# Autodesk Inventor assembly: Plastic Gear Test
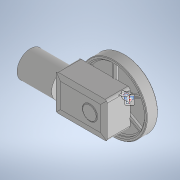
[picture p0: Inventor's stored thumbnail of the model, 180x180]
Saved by Autodesk Inventor 2020.2 (Build 242310000, 310)
## iProperties
Created: 2020-04-13
Part Number: Plastic Gear Test
Document SubType Name: Assembly
Designer: Josiah
Author: Josiah
## Documents named in this file (3)
- C:\Users\josia\OneDrive\Apps\0011_VentControlValve\Plastic Gear Test.iam
- C:\Users\josia\OneDrive\Apps\0011_VentControlValve\motor+Gearbox.ipt
- C:\Users\josia\OneDrive\Apps\0011_VentControlValve\Test Gear.ipt
## Components (2 placed, 2 different names)
1. motor+Gearbox:1 — Flush:1, Mate:1, Angle:1
2. Test Gear:1 — Flush:1, Mate:1, Angle:1
## Relationships (3: Flush 1, Mate 1, Angle 1)
- Flush:1: motor+Gearbox:1 ↔ Test Gear:1
- Mate:1: motor+Gearbox:1 ↔ Test Gear:1
- Angle:1 (180 deg): motor+Gearbox:1 ↔ Test Gear:1
